# Autodesk Inventor assembly: Robot
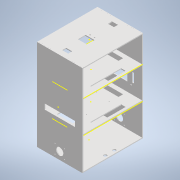
[picture p0: Inventor's stored thumbnail of the model, 180x180]
Saved by Autodesk Inventor 2020 (Build 240168000, 168)
## iProperties
Created: 2020-01-22
Part Number: Robot
Document SubType Name: Assembly
Designer: jelte
Mass: 570.337 g
Surface Area: 4038.22 cm^2
Volume: 570.337 cm^3
Density: 1 g/cm^3
Author: jelte
## Documents named in this file (7)
- E:\School\SJS 6EA-ICT\EAC\GIP\EA\3D Tekeningen\Robot.iam
- E:\School\SJS 6EA-ICT\EAC\GIP\EA\3D Tekeningen\MuurL.ipt
- E:\School\SJS 6EA-ICT\EAC\GIP\EA\3D Tekeningen\Level1 (motoren).ipt
- E:\School\SJS 6EA-ICT\EAC\GIP\EA\3D Tekeningen\Level2 (arduino).ipt
- E:\School\SJS 6EA-ICT\EAC\GIP\EA\3D Tekeningen\Level3 (voeding).ipt
- E:\School\SJS 6EA-ICT\EAC\GIP\EA\3D Tekeningen\Level4 (sensor + schakelaar).ipt
- E:\School\SJS 6EA-ICT\EAC\GIP\EA\3D Tekeningen\MuurR.ipt
## Components (6 placed, 6 different names)
1. Level2 (arduino):1
2. Level3 (voeding):1
3. Level1 (motoren):1
4. Level4 (sensor + schakelaar):1 — Rigid:8, Rigid:9
5. MuurR:1 — Rigid:8
6. MuurL:1 — Rigid:9
## Relationships (2: WeldJoint 2)
- Rigid:8 [WeldJoint]: Level4 (sensor + schakelaar):1 ↔ MuurR:1
- Rigid:9 [WeldJoint]: Level4 (sensor + schakelaar):1 ↔ MuurL:1
